# Autodesk Inventor assembly: FoldSlideLift
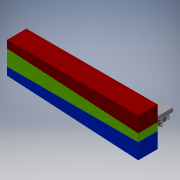
[picture p0: Inventor's stored thumbnail of the model, 180x180]
Saved by Autodesk Inventor 2017 (Build 210142000, 142)
## iProperties
Created: 2017-11-15
Part Number: FoldSlideLift
Document SubType Name: Assembly
Designer: User
Author: User
## Documents named in this file (5)
- C:\Robotics\CAD\2017-18_CAD\Prototypes\FoldSlideLift.iam
- C:\Robotics\CAD\2017-18_CAD\Prototypes\FoldLiftPart1.ipt
- C:\Robotics\CAD\COTSParts\Tetrix\Tetrix servo 180.ipt
- C:\Robotics\CAD\COTSParts\Tetrix\39060_txm-standard servo bracket.ipt
- C:\Robotics\CAD\2017-18_CAD\Prototypes\FoldSlidePart2.ipt
## Components (9 placed, 4 different names)
1. FoldLiftPart1:1 — Flush:2, Mate:6, Flush:5, Flush:8, Flush:10, Mate:15
2. FoldLiftPart1:2 — Flush:4, Mate:12, Flush:9, Mate:14
3. FoldLiftPart1:3 — Flush:2, Flush:4, Mate:8, Mate:14, Mate:15
4. Tetrix servo 180:1 — Mate:3, Mate:4, Mate:5, Mate:8
5. Tetrix servo 180:2 — Mate:9, Mate:10, Mate:11
6. 39060_txm-standard servo bracket:1 — Mate:3, Mate:4, Mate:5, Mate:7, Flush:7
7. 39060_txm-standard servo bracket:2 — Mate:9, Mate:10, Mate:11, Flush:11, Mate:13, Flush:12
8. FoldSlidePart2:1 — Mate:6, Flush:5, Mate:7, Flush:7, Flush:8
9. FoldSlidePart2:2 — Mate:12, Flush:9, Flush:10, Flush:11, Mate:13, Flush:12
## Relationships (22: Mate 13, Flush 9)
- Flush:2: FoldLiftPart1:1 ↔ FoldLiftPart1:3
- Flush:4: FoldLiftPart1:2 ↔ FoldLiftPart1:3
- Mate:3: Tetrix servo 180:1 ↔ 39060_txm-standard servo bracket:1
- Mate:4: Tetrix servo 180:1 ↔ 39060_txm-standard servo bracket:1
- Mate:5: Tetrix servo 180:1 ↔ 39060_txm-standard servo bracket:1
- Mate:6: FoldLiftPart1:1 ↔ FoldSlidePart2:1
- Flush:5: FoldLiftPart1:1 ↔ FoldSlidePart2:1
- Mate:7: 39060_txm-standard servo bracket:1 ↔ FoldSlidePart2:1
- Flush:7: 39060_txm-standard servo bracket:1 ↔ FoldSlidePart2:1
- Flush:8 (34.29 mm): FoldLiftPart1:1 ↔ FoldSlidePart2:1
- Mate:8: FoldLiftPart1:3 ↔ Tetrix servo 180:1
- Mate:9: Tetrix servo 180:2 ↔ 39060_txm-standard servo bracket:2
- Mate:10: Tetrix servo 180:2 ↔ 39060_txm-standard servo bracket:2
- Mate:11: Tetrix servo 180:2 ↔ 39060_txm-standard servo bracket:2
- Mate:12: FoldLiftPart1:2 ↔ FoldSlidePart2:2
- Flush:9: FoldLiftPart1:2 ↔ FoldSlidePart2:2
- Flush:10 (62.23 mm): FoldLiftPart1:1 ↔ FoldSlidePart2:2
- Flush:11: 39060_txm-standard servo bracket:2 ↔ FoldSlidePart2:2
- Mate:13: 39060_txm-standard servo bracket:2 ↔ FoldSlidePart2:2
- Flush:12: 39060_txm-standard servo bracket:2 ↔ FoldSlidePart2:2
- Mate:14: FoldLiftPart1:2 ↔ FoldLiftPart1:3
- Mate:15: FoldLiftPart1:1 ↔ FoldLiftPart1:3
